# Autodesk Inventor assembly: Ensamblaje4
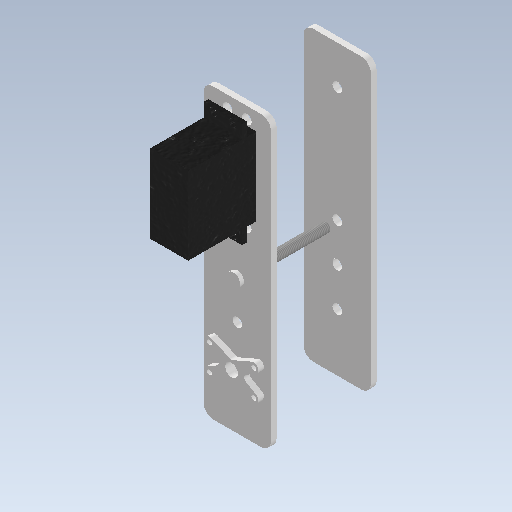
[picture p0: Inventor's stored thumbnail of the model, 512x512]
Saved by Autodesk Inventor 2021 (Build 250183000, 183)
## iProperties
Created: 2021-04-03
Part Number: Ensamblaje4
Document SubType Name: Assembly
Designer: diego
Author: diego
## Documents named in this file (6)
- C:\Users\diego\Desktop\Diego\Utadeo 2021-1\Robotica Industrial\Corte 2\Solido planos\Ensamblaje4.iam
- C:\Users\diego\Desktop\Diego\Utadeo 2021-1\Robotica Industrial\Corte 2\Solido planos\3.ipt
- C:\Users\diego\Desktop\Diego\Utadeo 2021-1\Robotica Industrial\Corte 2\Solido planos\Servo.ipt
- C:\Users\diego\Desktop\Diego\Utadeo 2021-1\Robotica Industrial\Corte 2\Solido planos\Extension2.ipt
- C:\Users\diego\Desktop\Diego\Utadeo 2021-1\Robotica Industrial\Corte 2\Solido planos\Tornillo_Corto.ipt
- C:\Users\diego\Desktop\Diego\Utadeo 2021-1\Robotica Industrial\Corte 2\Solido planos\4.ipt
## Components (5 placed, 5 different names)
1. 3:1 — De rotación:1, Insertar:1, Rígido:1
2. Servo:1 — De rotación:1
3. Extension2:1 — Insertar:1
4. Tornillo_Corto:1 — Rígido:1, Rígido:2, Rígido:3
5. 4:1 — Rígido:2, Rígido:3
## Relationships (5: WeldJoint 3, RevoluteJoint 1, Insert 1)
- De rotación:1 [RevoluteJoint] (3 mm): 3:1 ↔ Servo:1
- Insertar:1: 3:1 ↔ Extension2:1
- Rígido:1 [WeldJoint]: 3:1 ↔ Tornillo_Corto:1
- Rígido:2 [WeldJoint] (-12 mm): Tornillo_Corto:1 ↔ 4:1
- Rígido:3 [WeldJoint] (-15 mm): Tornillo_Corto:1 ↔ 4:1
